# Autodesk Inventor assembly: KON_Nietmaschine_gesamt
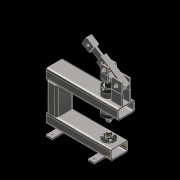
[picture p0: Inventor's stored thumbnail of the model, 180x180]
Saved by Autodesk Inventor 2019 (Build 230136000, 136)
## iProperties
Created: 2021-12-14
Part Number: KON_Nietmaschine_gesamt
Material: Generisch
Document SubType Name: Assembly
Designer: Jonas Nebl
Mass: 24988.3 g
Surface Area: 8290.64 cm^2
Volume: 3176.19 cm^3
Density: 7.86738 g/cm^3
Author: Jonas Nebl
## Documents named in this file (21)
- C:\Users\jonas\Documents\Inventor\Nietmaschine\KON_Nietmaschine_gesamt.iam
- C:\Users\jonas\Documents\Inventor\Nietmaschine\KON_Nietmaschine_Rahmen.iam
- C:\Users\jonas\Documents\Inventor\Nietmaschine\KON_Nietmaschine_Hebel.iam
- C:\Users\jonas\Documents\Inventor\Content Center Files\R2019\de-DE\DIN ISO 4379 F\DIN ISO 4379 - F 16 x 22 x 15.ipt
- C:\Users\jonas\Documents\Inventor\Nietmaschine\KON_Nietmaschine_Bolzen.ipt
- C:\Users\jonas\Documents\Inventor\Content Center Files\R2019\de-DE\DIN 471(2)\DIN 471 - 15 x 1(1).ipt
- C:\Users\jonas\Documents\Inventor\Nietmaschine\KON_Nietmaschine_Stempelwerkzeug_Matrize.ipt
- C:\Users\jonas\Documents\Inventor\Nietmaschine\KON_Nietmaschine_Schraubenfeder.ipt
- C:\Users\jonas\Documents\Inventor\Nietmaschine\KON_Nietmaschine_Dorn.iam
- C:\Users\jonas\Documents\Inventor\Nietmaschine\KON_Nietmaschine_Gleitstein.ipt
- C:\Users\jonas\Documents\Inventor\Nietmaschine\KON_Nietmaschine_Deckel.ipt
- C:\Users\jonas\Documents\Inventor\Nietmaschine\DIN EN 10220(2) - 57 x 5 - 100.ipt
- C:\Users\jonas\Documents\Inventor\Content Center Files\R2019\de-DE\DIN 912\DIN 912 - M5 x 0,8 x 20 x 18.ipt
- C:\Users\jonas\Documents\Inventor\Content Center Files\R2019\de-DE\DIN 472(1)\DIN 472 - 47 x 1,75.ipt
- C:\Users\jonas\Documents\Inventor\Content Center Files\R2019\de-DE\DIN 71412  A\DIN 71412 - AM 6 (kegelig kurz).ipt
- C:\Users\jonas\Documents\Inventor\Nietmaschine\Matrizenhalterung_unten.ipt
- C:\Users\jonas\Documents\Inventor\Nietmaschine\KON_Nietmaschine_Deckel_unten.ipt
- C:\Users\jonas\Documents\Inventor\Content Center Files\R2019\de-DE\DIN 913\DIN 913 - M4 x 8.ipt
- C:\Users\jonas\Documents\Inventor\Nietmaschine\ISO 4379 - 32 x 40 x 20C.ipt
- C:\Users\jonas\Documents\Inventor\Content Center Files\R2019\de-DE\ISO 4762(1)\DIN EN ISO 4762 - M6 x 12.ipt
- C:\Users\jonas\Documents\Inventor\Content Center Files\R2019\de-DE\DIN 988(1)\DIN 988 - S35 x 45.ipt
## Components (35 placed, 20 different names)
1. KON_Nietmaschine_Rahmen:1 [sub-assembly] — Passend:1, Passend:6, Passend:7, Passend:8, Passend:20, Winkel:2, Winkel:3, Winkel:4, Winkel:5, Einfügen:24
2. KON_Nietmaschine_Hebel:1 [sub-assembly] — Passend:1, Passend:2, Passend:3, Passend:4, Passend:5, Fluchtend:1, Passend:18
3. DIN ISO 4379 (Mit Flanschansatz) F 16 x 22 x 15:1 — Passend:2, Passend:4
4. DIN ISO 4379 (Mit Flanschansatz) F 16 x 22 x 15:2 — Passend:3, Passend:5, Passend:6
5. KON_Nietmaschine_Bolzen:1 — Passend:7, Passend:8, Passend:11, Passend:12, Einfügen:17, Winkel:6
6. DIN 471 > 9mm <= 300mm 15 x 1:1 — Passend:11, Passend:12
7. KON_Nietmaschine_Schraubenfeder:1 — Passend:16, Tangential:1
8. KON_Nietmaschine_Stempelwerkzeug_Matrize:2 — Einfügen:2, Passend:30, Tangential:3
9. KON_Nietmaschine_Dorn:1 [sub-assembly] — Passend:16, Einfügen:2, Passend:19, Passend:28, Tangential:1, Passend:29, Passend:32, Einfügen:22, Einfügen:28
10. KON_Nietmaschine_Gleitstein:1 — Fluchtend:1, Passend:18, Passend:19
11. KON_Nietmaschine_Bolzen:2 — Einfügen:19, Einfügen:22
12. DIN EN 10220(2) - 57 x 5 - 100:1 — Passend:20, Winkel:2, Passend:21, Passend:22, Passend:23, Passend:28, Einfügen:12, Einfügen:23
13. KON_Nietmaschine_Deckel:1 — Passend:21, Passend:22, Passend:23, Einfügen:4, Einfügen:5, Einfügen:6, Passend:26, Passend:27, Passend:29, Einfügen:8, Einfügen:21, Einfügen:29
14. DIN 912 - ersetzt durch DIN EN ISO 4762 M5 x 20:1 — Einfügen:4
15. DIN 912 - ersetzt durch DIN EN ISO 4762 M5 x 20:2 — Einfügen:5
16. DIN 912 - ersetzt durch DIN EN ISO 4762 M5 x 20:3 — Einfügen:6
17. DIN 472 47 x 1,75:1 — Passend:26, Passend:27
18. DIN 71412 A AM 6 (kegelig kurz):1 — Einfügen:8
19. Matrizenhalterung_unten:1 — Einfügen:11, Passend:31, Winkel:5, Einfügen:24, Einfügen:25, Einfügen:26, Einfügen:27
20. KON_Nietmaschine_Stempelwerkzeug_Matrize:3 — Einfügen:11, Passend:30, Tangential:2
21. KON_Nietmaschine_Deckel_unten:1 — Einfügen:12, Einfügen:14, Einfügen:16, Einfügen:20, Einfügen:23, Einfügen:30
22. DIN 71412 A AM 6 (kegelig kurz):2 — Einfügen:14, Winkel:3, Winkel:4
23. DIN 472 47 x 1,75:2 — Einfügen:16
24. DIN 71412 A AM 6 (kegelig kurz):3 — Einfügen:17
25. DIN 71412 A AM 6 (kegelig kurz):4 — Einfügen:19
26. DIN 913 M4 x 8:1 — Passend:31, Tangential:2
27. DIN 913 M4 x 8:2 — Passend:32, Tangential:3
28. ISO 4379 (Zylindrisch) 32 x 40 x 20:1 — Einfügen:20, Winkel:7
29. ISO 4379 (Zylindrisch) 32 x 40 x 20:2 — Einfügen:21, Winkel:8
30. DIN EN ISO 4762 M6 x 12:1 — Einfügen:25
31. DIN EN ISO 4762 M6 x 12:2 — Einfügen:27
32. DIN EN ISO 4762 M6 x 12:3 — Einfügen:26
33. DIN 471 > 9mm <= 300mm 15 x 1:2 — Einfügen:28
34. DIN 988 S35 x 45:1 — Einfügen:29
35. DIN 988 S35 x 45:2 — Einfügen:30
## Relationships (57: Mate 24, Insert 22, Angle 7, Tangent 3, Flush 1)
- Passend:1 [Mate]: KON_Nietmaschine_Rahmen:1 ↔ KON_Nietmaschine_Hebel:1
- Passend:2 [Mate]: KON_Nietmaschine_Hebel:1 ↔ DIN ISO 4379 (Mit Flanschansatz) F 16 x 22 x 15:1
- Passend:3 [Mate]: KON_Nietmaschine_Hebel:1 ↔ DIN ISO 4379 (Mit Flanschansatz) F 16 x 22 x 15:2
- Passend:4 [Mate]: KON_Nietmaschine_Hebel:1 ↔ DIN ISO 4379 (Mit Flanschansatz) F 16 x 22 x 15:1
- Passend:5 [Mate]: KON_Nietmaschine_Hebel:1 ↔ DIN ISO 4379 (Mit Flanschansatz) F 16 x 22 x 15:2
- Passend:6 [Mate]: KON_Nietmaschine_Rahmen:1 ↔ DIN ISO 4379 (Mit Flanschansatz) F 16 x 22 x 15:2
- Passend:7 [Mate]: KON_Nietmaschine_Rahmen:1 ↔ KON_Nietmaschine_Bolzen:1
- Passend:8 [Mate] (-1 mm): KON_Nietmaschine_Rahmen:1 ↔ KON_Nietmaschine_Bolzen:1
- Passend:11 [Mate]: KON_Nietmaschine_Bolzen:1 ↔ DIN 471 > 9mm <= 300mm 15 x 1:1
- Passend:12 [Mate]: KON_Nietmaschine_Bolzen:1 ↔ DIN 471 > 9mm <= 300mm 15 x 1:1
- Passend:16 [Mate]: KON_Nietmaschine_Schraubenfeder:1 ↔ KON_Nietmaschine_Dorn:1
- Einfügen:2 [Insert]: KON_Nietmaschine_Stempelwerkzeug_Matrize:2 ↔ KON_Nietmaschine_Dorn:1
- Fluchtend:1 [Flush] (-3 mm): KON_Nietmaschine_Hebel:1 ↔ KON_Nietmaschine_Gleitstein:1
- Passend:18 [Mate]: KON_Nietmaschine_Hebel:1 ↔ KON_Nietmaschine_Gleitstein:1
- Passend:19 [Mate]: KON_Nietmaschine_Dorn:1 ↔ KON_Nietmaschine_Gleitstein:1
- Passend:20 [Mate]: KON_Nietmaschine_Rahmen:1 ↔ DIN EN 10220(2) - 57 x 5 - 100:1
- Winkel:2 [Angle] (210 deg): KON_Nietmaschine_Rahmen:1 ↔ DIN EN 10220(2) - 57 x 5 - 100:1
- Passend:21 [Mate]: DIN EN 10220(2) - 57 x 5 - 100:1 ↔ KON_Nietmaschine_Deckel:1
- Passend:22 [Mate]: DIN EN 10220(2) - 57 x 5 - 100:1 ↔ KON_Nietmaschine_Deckel:1
- Passend:23 [Mate]: DIN EN 10220(2) - 57 x 5 - 100:1 ↔ KON_Nietmaschine_Deckel:1
- Einfügen:4 [Insert]: KON_Nietmaschine_Deckel:1 ↔ DIN 912 - ersetzt durch DIN EN ISO 4762 M5 x 20:1
- Einfügen:5 [Insert]: KON_Nietmaschine_Deckel:1 ↔ DIN 912 - ersetzt durch DIN EN ISO 4762 M5 x 20:2
- Einfügen:6 [Insert]: KON_Nietmaschine_Deckel:1 ↔ DIN 912 - ersetzt durch DIN EN ISO 4762 M5 x 20:3
- Passend:26 [Mate]: KON_Nietmaschine_Deckel:1 ↔ DIN 472 47 x 1,75:1
- Passend:27 [Mate]: KON_Nietmaschine_Deckel:1 ↔ DIN 472 47 x 1,75:1
- Passend:28 [Mate]: KON_Nietmaschine_Dorn:1 ↔ DIN EN 10220(2) - 57 x 5 - 100:1
- Tangential:1: KON_Nietmaschine_Schraubenfeder:1 ↔ KON_Nietmaschine_Dorn:1
- Passend:29 [Mate]: KON_Nietmaschine_Dorn:1 ↔ KON_Nietmaschine_Deckel:1
- Einfügen:8 [Insert]: KON_Nietmaschine_Deckel:1 ↔ DIN 71412 A AM 6 (kegelig kurz):1
- Einfügen:11 [Insert]: Matrizenhalterung_unten:1 ↔ KON_Nietmaschine_Stempelwerkzeug_Matrize:3
- Einfügen:12 [Insert]: DIN EN 10220(2) - 57 x 5 - 100:1 ↔ KON_Nietmaschine_Deckel_unten:1
- Einfügen:14 [Insert]: KON_Nietmaschine_Deckel_unten:1 ↔ DIN 71412 A AM 6 (kegelig kurz):2
- Winkel:3 [Angle] (180 deg): KON_Nietmaschine_Rahmen:1 ↔ DIN 71412 A AM 6 (kegelig kurz):2
- Winkel:4 [Angle] (180 deg): KON_Nietmaschine_Rahmen:1 ↔ DIN 71412 A AM 6 (kegelig kurz):2
- Passend:30 [Mate] (50 mm): KON_Nietmaschine_Stempelwerkzeug_Matrize:2 ↔ KON_Nietmaschine_Stempelwerkzeug_Matrize:3
- Einfügen:16 [Insert]: KON_Nietmaschine_Deckel_unten:1 ↔ DIN 472 47 x 1,75:2
- Einfügen:17 [Insert]: KON_Nietmaschine_Bolzen:1 ↔ DIN 71412 A AM 6 (kegelig kurz):3
- Einfügen:19 [Insert]: KON_Nietmaschine_Bolzen:2 ↔ DIN 71412 A AM 6 (kegelig kurz):4
- Passend:31 [Mate]: Matrizenhalterung_unten:1 ↔ DIN 913 M4 x 8:1
- Tangential:2: KON_Nietmaschine_Stempelwerkzeug_Matrize:3 ↔ DIN 913 M4 x 8:1
- Passend:32 [Mate]: KON_Nietmaschine_Dorn:1 ↔ DIN 913 M4 x 8:2
- Tangential:3: KON_Nietmaschine_Stempelwerkzeug_Matrize:2 ↔ DIN 913 M4 x 8:2
- Winkel:5 [Angle] (0 deg): KON_Nietmaschine_Rahmen:1 ↔ Matrizenhalterung_unten:1
- Einfügen:20 [Insert]: KON_Nietmaschine_Deckel_unten:1 ↔ ISO 4379 (Zylindrisch) 32 x 40 x 20:1
- Einfügen:21 [Insert]: KON_Nietmaschine_Deckel:1 ↔ ISO 4379 (Zylindrisch) 32 x 40 x 20:2
- Einfügen:22 [Insert]: KON_Nietmaschine_Dorn:1 ↔ KON_Nietmaschine_Bolzen:2
- Winkel:6 [Angle] (0 deg): KON_Nietmaschine_Bolzen:1
- Winkel:7 [Angle] (0 deg): ISO 4379 (Zylindrisch) 32 x 40 x 20:1
- Winkel:8 [Angle] (0 deg): ISO 4379 (Zylindrisch) 32 x 40 x 20:2
- Einfügen:23 [Insert]: DIN EN 10220(2) - 57 x 5 - 100:1 ↔ KON_Nietmaschine_Deckel_unten:1
- Einfügen:24 [Insert]: KON_Nietmaschine_Rahmen:1 ↔ Matrizenhalterung_unten:1
- Einfügen:25 [Insert]: Matrizenhalterung_unten:1 ↔ DIN EN ISO 4762 M6 x 12:1
- Einfügen:26 [Insert]: Matrizenhalterung_unten:1 ↔ DIN EN ISO 4762 M6 x 12:3
- Einfügen:27 [Insert]: Matrizenhalterung_unten:1 ↔ DIN EN ISO 4762 M6 x 12:2
- Einfügen:28 [Insert]: KON_Nietmaschine_Dorn:1 ↔ DIN 471 > 9mm <= 300mm 15 x 1:2
- Einfügen:29 [Insert]: KON_Nietmaschine_Deckel:1 ↔ DIN 988 S35 x 45:1
- Einfügen:30 [Insert]: KON_Nietmaschine_Deckel_unten:1 ↔ DIN 988 S35 x 45:2
